# Autodesk Inventor assembly: wheel
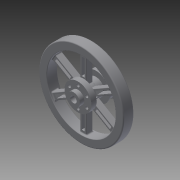
[picture p0: Inventor's stored thumbnail of the model, 180x180]
Saved by Autodesk Inventor 2015 (Build 190159000, 159)
## iProperties
Created: 2015-07-19
Part Number: wheel
Document SubType Name: Assembly
Designer: astralien3000
Author: astralien3000
## Documents named in this file (4)
- C:\Users\astralien3000\Desktop\ceres\meca\v2016\wheel.iam
- C:\Users\astralien3000\Desktop\ceres\meca\lib\wheel\pololu_wheel_80x10.ipt
- C:\Users\astralien3000\Desktop\ceres\meca\lib\struct\hub_6mm_M3.ipt
- C:\Users\astralien3000\Desktop\ceres\meca\lib\struct\poulie_conrad_209515.ipt
## Components (3 placed, 3 different names)
1. pololu_wheel_80x10:1 — Placage:1, Placage:2, Placage:3, Placage:4, Placage:7, Placage:8
2. hub_6mm_M3:1 — Placage:3, Placage:4
3. poulie_conrad_209515:1 — Placage:7, Placage:8
## Relationships (6: Mate 6)
- Placage:1 [Mate]: pololu_wheel_80x10:1
- Placage:2 [Mate]: pololu_wheel_80x10:1
- Placage:3 [Mate]: pololu_wheel_80x10:1 ↔ hub_6mm_M3:1
- Placage:4 [Mate]: pololu_wheel_80x10:1 ↔ hub_6mm_M3:1
- Placage:7 [Mate]: pololu_wheel_80x10:1 ↔ poulie_conrad_209515:1
- Placage:8 [Mate]: pololu_wheel_80x10:1 ↔ poulie_conrad_209515:1
